# Autodesk Inventor assembly: C板转配体
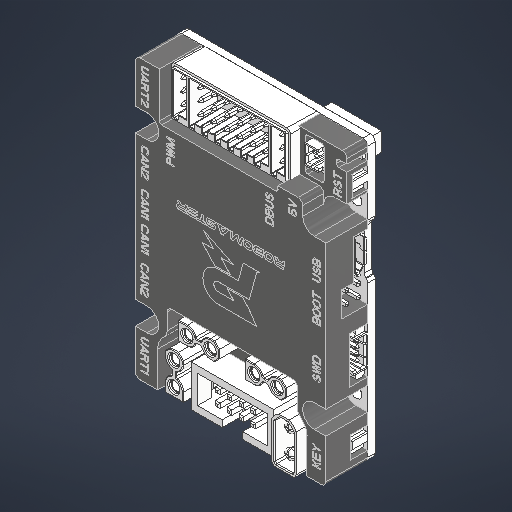
[picture p0: Inventor's stored thumbnail of the model, 512x512]
Saved by Autodesk Inventor 2025 (Build 290162000, 162)
## iProperties
Created: 2024-07-05
Part Number: C板转配体
Document SubType Name: Assembly
Designer: HZD
Author: HZD
## Documents named in this file (5)
- D:\2 B Mechanical design\GCG全向轮步兵\云台\C板转配体.iam
- D:\2 B Mechanical design\GCG全向轮步兵\云台\1_0.stp.ipt
- D:\2 B Mechanical design\GCG全向轮步兵\云台\2_0.stp.ipt
- 1_0.stp
- 2_0.stp
## Components (2 placed, 2 different names)
1. 1_0.stp:1 — 配合:3, 表面齐平:1
2. 2_0.stp:1 — 配合:3, 表面齐平:1
## Relationships (2: Mate 1, Flush 1)
- 配合:3 [Mate]: 1_0.stp:1 ↔ 2_0.stp:1
- 表面齐平:1 [Flush]: 1_0.stp:1 ↔ 2_0.stp:1
